# Autodesk Inventor assembly: UNIVERSAL JOINT
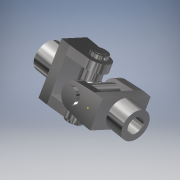
[picture p0: Inventor's stored thumbnail of the model, 180x180]
Saved by Autodesk Inventor 2018 (Build 220112000, 112)
## iProperties
Created: 2018-09-13
Part Number: UNIVERSAL JOINT
Document SubType Name: Assembly
Designer: Ajay Sharma
Author: Ajay Sharma
## Documents named in this file (5)
- C:\Users\Ajay Sharma\Documents\UNIVERSAL JOINT.iam
- C:\Users\Ajay Sharma\Documents\Fork 2 Off.ipt
- C:\Users\Ajay Sharma\Documents\Centre Block.ipt
- C:\Users\Ajay Sharma\Documents\Pin.ipt
- C:\Users\Ajay Sharma\Documents\Collar 2.ipt
## Components (7 placed, 4 different names)
1. Fork 2 Off:1 — Mate:1, Mate:2, Mate:4, Mate:13
2. Fork 2 Off:2 — Mate:5, Mate:6, Mate:8, Mate:13
3. Centre Block:1 — Mate:3, Mate:4, Mate:7, Mate:8
4. Pin:1 — Mate:1, Mate:2, Mate:3, Mate:11, Mate:12
5. Pin:2 — Mate:5, Mate:6, Mate:7, Mate:9, Mate:10
6. Collar 2:1 — Mate:9, Mate:10
7. Collar 2:2 — Mate:11, Mate:12
## Relationships (13: Mate 13)
- Mate:1: Fork 2 Off:1 ↔ Pin:1
- Mate:2: Fork 2 Off:1 ↔ Pin:1
- Mate:3: Centre Block:1 ↔ Pin:1
- Mate:4: Fork 2 Off:1 ↔ Centre Block:1
- Mate:5: Fork 2 Off:2 ↔ Pin:2
- Mate:6: Fork 2 Off:2 ↔ Pin:2
- Mate:7: Centre Block:1 ↔ Pin:2
- Mate:8: Fork 2 Off:2 ↔ Centre Block:1
- Mate:9: Pin:2 ↔ Collar 2:1
- Mate:10: Pin:2 ↔ Collar 2:1
- Mate:11: Pin:1 ↔ Collar 2:2
- Mate:12: Pin:1 ↔ Collar 2:2
- Mate:13: Fork 2 Off:1 ↔ Fork 2 Off:2
